# Autodesk Inventor assembly: Full Landing Docks Third Iteration
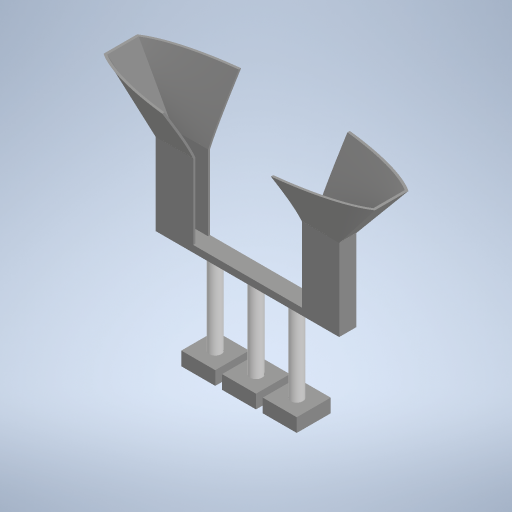
[picture p0: Inventor's stored thumbnail of the model, 512x512]
Saved by Autodesk Inventor 2023 (Build 270158000, 158)
## iProperties
Created: 2023-02-22
Part Number: Full Landing Docks Third Iteration
Document SubType Name: Assembly
Designer: mihal
Author: mihal
## Documents named in this file (4)
- C:\Users\mihal\Desktop\4th Year Project\Final Assembly\Landing Docks\Full Landing Docks.iam
- C:\Users\mihal\Desktop\4th Year Project\Final Assembly\Landing Docks\Base of Landing Docks.ipt
- C:\Users\mihal\Desktop\4th Year Project\Final Assembly\Landing Docks\Landing Docks Funnel .ipt
- C:\Users\mihal\Desktop\4th Year Project\Final Assembly\Landing Docks\Landing Dock Legs.ipt
## Components (8 placed, 3 different names)
1. Base of Landing Docks:1 — Mate:1, Mate:2
2. Landing Docks Funnel :1 — Mate:16, Mate:17, Mate:18, Mate:19, Mate:20, Mate:21
3. Landing Dock Legs:1 — Mate:1, Mate:2, Mate:11, Mate:12, Mate:18, Mate:19
4. Landing Dock Legs:2 — Mate:9, Mate:10, Mate:16, Mate:17
5. Landing Dock Legs:3 — Mate:13, Mate:14, Mate:20, Mate:21
6. Base of Landing Docks:2 — Mate:13, Mate:14, Flush:2
7. Base of Landing Docks:3 — Mate:11, Mate:12, Flush:1, Flush:2
8. Base of Landing Docks:4 — Mate:9, Mate:10, Flush:1, Mate:22
## Relationships (17: Mate 15, Flush 2)
- Mate:1: Base of Landing Docks:1 ↔ Landing Dock Legs:1
- Mate:2: Base of Landing Docks:1 ↔ Landing Dock Legs:1
- Mate:9: Landing Dock Legs:2 ↔ Base of Landing Docks:4
- Mate:10: Landing Dock Legs:2 ↔ Base of Landing Docks:4
- Mate:11: Landing Dock Legs:1 ↔ Base of Landing Docks:3
- Mate:12: Landing Dock Legs:1 ↔ Base of Landing Docks:3
- Mate:13: Landing Dock Legs:3 ↔ Base of Landing Docks:2
- Mate:14: Landing Dock Legs:3 ↔ Base of Landing Docks:2
- Mate:16: Landing Docks Funnel :1 ↔ Landing Dock Legs:2
- Mate:17: Landing Docks Funnel :1 ↔ Landing Dock Legs:2
- Mate:18: Landing Docks Funnel :1 ↔ Landing Dock Legs:1
- Mate:19: Landing Docks Funnel :1 ↔ Landing Dock Legs:1
- Mate:20: Landing Docks Funnel :1 ↔ Landing Dock Legs:3
- Mate:21: Landing Docks Funnel :1 ↔ Landing Dock Legs:3
- Flush:1: Base of Landing Docks:3 ↔ Base of Landing Docks:4
- Flush:2: Base of Landing Docks:2 ↔ Base of Landing Docks:3
- Mate:22: Base of Landing Docks:4
